# Autodesk Inventor assembly: chess_assembly
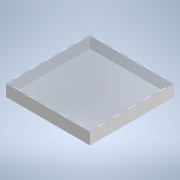
[picture p0: Inventor's stored thumbnail of the model, 180x180]
Saved by Autodesk Inventor 2020 (Build 240168000, 168)
## iProperties
Created: 2020-03-10
Part Number: chess_assembly
Document SubType Name: Assembly
Designer: udvarhelyi
Author: udvarhelyi
## Documents named in this file (3)
- C:\Users\udvarhelyi\Desktop\Escape_2020\Escape_chess\chess_assembly.iam
- C:\Users\udvarhelyi\Desktop\Escape_2020\Escape_chess\base.ipt
- C:\Users\udvarhelyi\Desktop\Escape_2020\Escape_chess\side.ipt
## Components (6 placed, 2 different names)
1. base:1 — Flush:1, Mate:1, Flush:2, Flush:3, Flush:5, Flush:6, Flush:8, Flush:9, Flush:10
2. side:1 — Flush:1, Mate:1, Flush:2, Flush:4, Flush:7, Flush:12, Flush:13
3. side:3 — Flush:3, Flush:4, Flush:5
4. side:4 — Flush:9, Flush:10, Flush:11
5. side:5 — Flush:6, Flush:7, Flush:8, Flush:11, Flush:14
6. base:2 — Flush:12, Flush:13, Flush:14
## Relationships (15: Flush 14, Mate 1)
- Flush:1: base:1 ↔ side:1
- Mate:1: base:1 ↔ side:1
- Flush:2: base:1 ↔ side:1
- Flush:3: base:1 ↔ side:3
- Flush:4: side:1 ↔ side:3
- Flush:5: base:1 ↔ side:3
- Flush:6: base:1 ↔ side:5
- Flush:7: side:1 ↔ side:5
- Flush:8: base:1 ↔ side:5
- Flush:9: base:1 ↔ side:4
- Flush:10: base:1 ↔ side:4
- Flush:11: side:4 ↔ side:5
- Flush:12: side:1 ↔ base:2
- Flush:13: side:1 ↔ base:2
- Flush:14: side:5 ↔ base:2
